# Autodesk Inventor assembly: 4 Omni, Circle_MIR
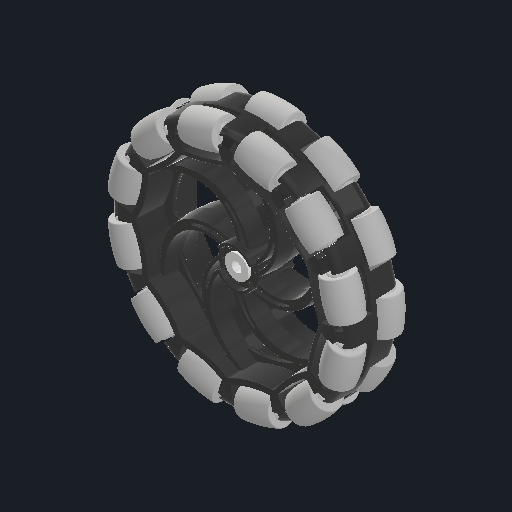
[picture p0: Inventor's stored thumbnail of the model, 512x512]
Saved by Autodesk Inventor 2024 (Build 280153000, 153)
## iProperties
Created: 2022-08-02
Part Number: 4 Omni, Circle_MIR
Document SubType Name: Assembly
Designer: macbook
Author: ylu12
## Documents named in this file (3)
- \\Mac\Home\Desktop\code\7899V-VRC-OVER-UNDER\Cad\VEX-CAD-Inventor-1.4.0\Motion\Wheels\Omni Wheel\4 Omni, Circle_MIR.iam
- \\Mac\Home\Desktop\code\7899V-VRC-OVER-UNDER\Cad\VEX-CAD-Inventor-1.4.0\Motion\Wheels\Reference Files\4 Omni_MIR.ipt
- \\Mac\Home\Desktop\code\7899V-VRC-OVER-UNDER\Cad\VEX-CAD-Inventor-1.4.0\Motion\Insert Circle_MIR.ipt
## Components (3 placed, 2 different names)
1. 4 Omni_MIR:1 — Flush:8, Mate:16, Mate:15
2. Insert Circle_MIR:1 — Angle:2, Mate:20, Flush:13, Flush:12, Flush:14
3. Insert Circle_MIR:2 — Flush:13, Flush:12, Mate:19
## Relationships (9: Flush 4, Mate 4, Angle 1)
- Flush:8: 4 Omni_MIR:1
- Mate:16: 4 Omni_MIR:1
- Mate:15: 4 Omni_MIR:1
- Angle:2 (0 deg): Insert Circle_MIR:1
- Mate:20: Insert Circle_MIR:1
- Flush:13: Insert Circle_MIR:1 ↔ Insert Circle_MIR:2
- Flush:12: Insert Circle_MIR:1 ↔ Insert Circle_MIR:2
- Flush:14 [Mate] (7.0104 mm): Insert Circle_MIR:1
- Mate:19 [Flush] (7.0104 mm): Insert Circle_MIR:2
